# Autodesk Inventor assembly: End Ramp Assembly
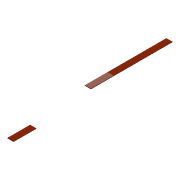
[picture p0: Inventor's stored thumbnail of the model, 180x180]
Saved by Autodesk Inventor 2015 (Build 190159000, 159)
## iProperties
Created: 2015-01-20
Part Number: End Ramp Assembly
Document SubType Name: Assembly
Designer: Peter
Author: Peter
## Documents named in this file (5)
- T:\FILES\FIRST-Team-1719-CAD-Team\2015 Playing Field\Team 1719 Practice Field\Scoring Platform - Construction Design\End Ramp Assembly.iam
- T:\FILES\FIRST-Team-1719-CAD-Team\2015 Playing Field\Team 1719 Practice Field\Scoring Platform - Construction Design\Clear Ramp Surface 125 - Version 2.ipt
- T:\FILES\FIRST-Team-1719-CAD-Team\2015 Playing Field\Team 1719 Practice Field\Scoring Platform - Construction Design\Plywood Ramp 375 - Versopm 2.ipt
- T:\FILES\FIRST-Team-1719-CAD-Team\2015 Playing Field\Team 1719 Practice Field\Scoring Platform - Construction Design\End Plywood Ramp 375.ipt
- T:\FILES\FIRST-Team-1719-CAD-Team\2015 Playing Field\Team 1719 Practice Field\Scoring Platform - Construction Design\End Clear Ramp Surface 125 - Version 2.ipt
## Components (4 placed, 4 different names)
1. Clear Ramp Surface 125 - Version 2:1 — Mate:1, Flush:1, Flush:2
2. Plywood Ramp 375 - Versopm 2:1 — Mate:1, Flush:1, Flush:2
3. End Plywood Ramp 375:1 — Mate:2, Flush:3, Flush:4
4. End Clear Ramp Surface 125 - Version 2:1 — Mate:2, Flush:3, Flush:4
## Relationships (6: Flush 4, Mate 2)
- Mate:1: Clear Ramp Surface 125 - Version 2:1 ↔ Plywood Ramp 375 - Versopm 2:1
- Flush:1: Clear Ramp Surface 125 - Version 2:1 ↔ Plywood Ramp 375 - Versopm 2:1
- Flush:2: Clear Ramp Surface 125 - Version 2:1 ↔ Plywood Ramp 375 - Versopm 2:1
- Mate:2: End Plywood Ramp 375:1 ↔ End Clear Ramp Surface 125 - Version 2:1
- Flush:3: End Plywood Ramp 375:1 ↔ End Clear Ramp Surface 125 - Version 2:1
- Flush:4: End Plywood Ramp 375:1 ↔ End Clear Ramp Surface 125 - Version 2:1
